# Autodesk Inventor assembly: gripper_base_frame
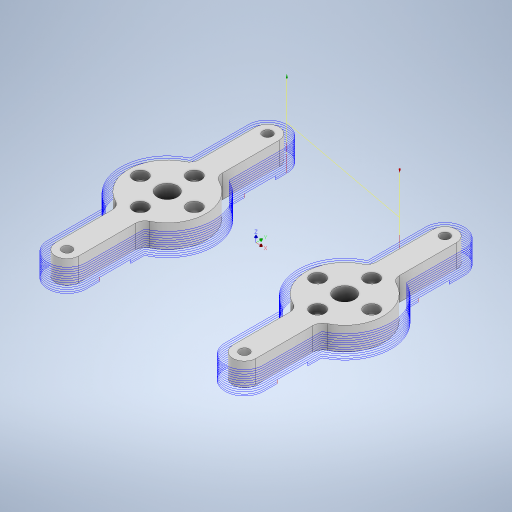
[picture p0: Inventor's stored thumbnail of the model, 512x512]
Saved by Autodesk Inventor 2024.2 (Build 282272000, 272)
## iProperties
Created: 2024-01-10
Part Number: gripper_base_frame
Document SubType Name: Assembly
Designer: chanh
Author: chanh
## Documents named in this file (2)
- C:\Users\chanh\내 드라이브\로봇\Humanoid\Roboin Humanoid Project\Inventor\rh_plus_7_axis_robot_arm_hardware\CAM\6T\gripper_base_frame.iam
- C:\Users\chanh\내 드라이브\로봇\Humanoid\Roboin Humanoid Project\Inventor\rh_plus_7_axis_robot_arm_hardware\CAM\6T\gripper_base_frame.ipt
## Components (2 placed, 1 different names)
1. gripper_base_frame:1 — Mate:1, Flush:1, Flush:2, Mate:2, Flush:3, Flush:4
2. gripper_base_frame:2 — Mate:2, Flush:3, Flush:4
## Relationships (6: Flush 4, Mate 2)
- Mate:1: gripper_base_frame:1
- Flush:1: gripper_base_frame:1
- Flush:2: gripper_base_frame:1
- Mate:2 (40 mm): gripper_base_frame:1 ↔ gripper_base_frame:2
- Flush:3: gripper_base_frame:1 ↔ gripper_base_frame:2
- Flush:4: gripper_base_frame:1 ↔ gripper_base_frame:2
